# Autodesk Inventor assembly: 装配-主动轮
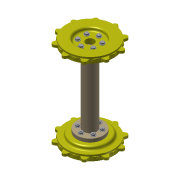
[picture p0: Inventor's stored thumbnail of the model, 180x180]
Saved by Autodesk Inventor 2015 (Build 190159000, 159)
## iProperties
Created: 2017-05-23
Part Number: 装配-主动轮
Document SubType Name: Assembly
Designer: Administrator
Author: Administrator
## Documents named in this file (5)
- C:\Users\Administrator\Desktop\毕设改终\装配-主动轮.iam
- C:\Users\Administrator\Desktop\毕设改终\主动轮.ipt
- C:\Users\Administrator\Desktop\毕设改终\主动轮固定螺帽.ipt
- C:\Users\Administrator\Desktop\毕设改终\主动轮固定螺丝.ipt
- C:\Users\Administrator\Desktop\毕设改终\主动轮连接筒.ipt
## Components (27 placed, 4 different names)
1. 主动轮:1 — 插入:1, 插入:2, 插入:5
2. 主动轮:2 — 插入:9, 插入:10
3. 主动轮连接筒:1 — 插入:1, 插入:2, 插入:6, 插入:8, 插入:9, 插入:10
4. 主动轮固定螺丝:1 — 插入:5
5. 主动轮固定螺帽:1 — 插入:6
6. 主动轮固定螺帽:2 — 插入:8
7. 主动轮固定螺丝:2
8. 主动轮固定螺丝:3
9. 主动轮固定螺帽:3
10. 主动轮固定螺帽:4
11. 主动轮固定螺丝:4
12. 主动轮固定螺丝:5
13. 主动轮固定螺帽:5
14. 主动轮固定螺帽:6
15. 主动轮固定螺丝:6
16. 主动轮固定螺丝:7
17. 主动轮固定螺帽:7
18. 主动轮固定螺帽:8
19. 主动轮固定螺丝:8
20. 主动轮固定螺丝:9
21. 主动轮固定螺帽:9
22. 主动轮固定螺帽:10
23. 主动轮固定螺丝:10
24. 主动轮固定螺丝:11
25. 主动轮固定螺帽:11
26. 主动轮固定螺帽:12
27. 主动轮固定螺丝:12
## Component patterns: (6 elements, first: 主动轮固定螺丝:1 + 主动轮固定螺帽:1 + 主动轮固定螺帽:2 + 主动轮固定螺丝:2)
## Relationships (7: Insert 7)
- 插入:1 [Insert]: 主动轮:1 ↔ 主动轮连接筒:1
- 插入:2 [Insert]: 主动轮:1 ↔ 主动轮连接筒:1
- 插入:5 [Insert]: 主动轮:1 ↔ 主动轮固定螺丝:1
- 插入:6 [Insert]: 主动轮连接筒:1 ↔ 主动轮固定螺帽:1
- 插入:8 [Insert]: 主动轮连接筒:1 ↔ 主动轮固定螺帽:2
- 插入:9 [Insert]: 主动轮:2 ↔ 主动轮连接筒:1
- 插入:10 [Insert]: 主动轮:2 ↔ 主动轮连接筒:1
